# Autodesk Inventor assembly: BowdenDriver
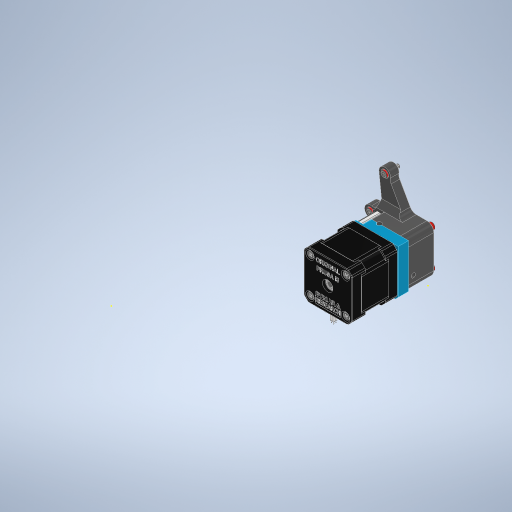
[picture p0: Inventor's stored thumbnail of the model, 512x512]
Saved by Autodesk Inventor 2023 (Build 270158000, 158)
## iProperties
Created: 2023-06-16
Part Number: BowdenDriver
Document SubType Name: Assembly
Designer: Parker
Author: Parker
## Documents named in this file (13)
- D:\000 - PEPCORP CLOUD\00- Legacy\Designs\MK3PRO P1\E2\BowdenDriver.iam
- D:\000 - PEPCORP CLOUD\00- Legacy\Designs\MK3PRO P1\E2\Bowden Back.ipt
- D:\000 - PEPCORP CLOUD\00- Legacy\Designs\MK3PRO P1\E2\E-Motor Mount P1.1.ipt
- D:\000 - PEPCORP CLOUD\00- Legacy\Designs\MK3PRO P1\E2\Extruder Idler V3.ipt
- D:\000 - PEPCORP CLOUD\00- Legacy\Designs\MK3PRO P1\COMPONENTS\NUT_SQUARE_M3.ipt
- D:\000 - PEPCORP CLOUD\00- Legacy\Designs\MK3PRO P1\COMPONENTS\SHCS_M3_40.ipt
- D:\000 - PEPCORP CLOUD\00- Legacy\Designs\MK3PRO P1\COMPONENTS\M3 Washer.ipt
- D:\000 - PEPCORP CLOUD\00- Legacy\Designs\MK3PRO P1\COMPONENTS\Bondtech Idler.ipt
- D:\000 - PEPCORP CLOUD\00- Legacy\Designs\MK3PRO P1\E-Axis\Extruder_stepper_motor V2.iam
- D:\000 - PEPCORP CLOUD\00- Legacy\Designs\MK3PRO P1\COMPONENTS\Bondtech Driver.ipt
- D:\000 - PEPCORP CLOUD\00- Legacy\Designs\MK3PRO P1\COMPONENTS\SHCS_M3_35.ipt
- D:\000 - PEPCORP CLOUD\00- Legacy\Designs\MK3PRO P1\COMPONENTS\SHCS_M3_30.ipt
- D:\000 - PEPCORP CLOUD\00- Legacy\Designs\MK3PRO P1\COMPONENTS\SHCS_M3_8.ipt
## Components (16 placed, 12 different names)
1. Bowden Back:1 — Mate:1, Mate:2, Mate:3, Mate:4, Mate:5, Mate:6, Mate:7, Mate:8, Mate:15, Mate:16, Mate:18, Mate:19, Mate:20, Mate:21, Mate:22, Mate:23, Mate:24, Mate:25, Mate:26, Mate:27, Mate:28, Mate:29
2. E-Motor Mount P1.1:1 — Mate:1, Mate:2, Mate:3, Mate:14
3. Extruder Idler V3:1 — Mate:4, Mate:5, Mate:11, Mate:13, Flush:2
4. NUT_SQUARE_M3:1 — Mate:6, Mate:7, Flush:1
5. SHCS_M3_40:1 — Mate:8, Flush:1, Mate:9, Mate:10, Mate:12
6. M3 Washer:1 — Mate:9, Mate:10
7. M3 Washer:2 — Mate:11, Mate:12
8. Bondtech Idler:1 — Mate:13, Flush:2, Flush:3
9. Extruder_stepper_motor V2:1 [sub-assembly] — Mate:14, Mate:15, Mate:16, Mate:17
10. Bondtech Driver:1 — Mate:17, Flush:3
11. SHCS_M3_35:1 — Mate:20, Mate:22
12. SHCS_M3_35:2 — Mate:19, Mate:21
13. SHCS_M3_35:3 — Mate:18, Mate:23
14. SHCS_M3_30:1 — Mate:24, Mate:25
15. SHCS_M3_8:1 — Mate:26, Mate:29
16. SHCS_M3_8:2 — Mate:27, Mate:28
## Relationships (32: Mate 29, Flush 3)
- Mate:1: Bowden Back:1 ↔ E-Motor Mount P1.1:1
- Mate:2: Bowden Back:1 ↔ E-Motor Mount P1.1:1
- Mate:3: Bowden Back:1 ↔ E-Motor Mount P1.1:1
- Mate:4: Bowden Back:1 ↔ Extruder Idler V3:1
- Mate:5 (0.25 mm): Bowden Back:1 ↔ Extruder Idler V3:1
- Mate:6: Bowden Back:1 ↔ NUT_SQUARE_M3:1
- Mate:7: Bowden Back:1 ↔ NUT_SQUARE_M3:1
- Mate:8: Bowden Back:1 ↔ SHCS_M3_40:1
- Flush:1 (-5 mm): NUT_SQUARE_M3:1 ↔ SHCS_M3_40:1
- Mate:9: SHCS_M3_40:1 ↔ M3 Washer:1
- Mate:10: SHCS_M3_40:1 ↔ M3 Washer:1
- Mate:11: Extruder Idler V3:1 ↔ M3 Washer:2
- Mate:12: SHCS_M3_40:1 ↔ M3 Washer:2
- Mate:13: Extruder Idler V3:1 ↔ Bondtech Idler:1
- Flush:2 (1.5 mm): Extruder Idler V3:1 ↔ Bondtech Idler:1
- Mate:14: E-Motor Mount P1.1:1 ↔ Extruder_stepper_motor V2:1
- Mate:15: Bowden Back:1 ↔ Extruder_stepper_motor V2:1
- Mate:16: Bowden Back:1 ↔ Extruder_stepper_motor V2:1
- Mate:17: Extruder_stepper_motor V2:1 ↔ Bondtech Driver:1
- Flush:3: Bondtech Idler:1 ↔ Bondtech Driver:1
- Mate:18: Bowden Back:1 ↔ SHCS_M3_35:3
- Mate:19: Bowden Back:1 ↔ SHCS_M3_35:2
- Mate:20: Bowden Back:1 ↔ SHCS_M3_35:1
- Mate:21: Bowden Back:1 ↔ SHCS_M3_35:2
- Mate:22: Bowden Back:1 ↔ SHCS_M3_35:1
- Mate:23: Bowden Back:1 ↔ SHCS_M3_35:3
- Mate:24: Bowden Back:1 ↔ SHCS_M3_30:1
- Mate:25: Bowden Back:1 ↔ SHCS_M3_30:1
- Mate:26: Bowden Back:1 ↔ SHCS_M3_8:1
- Mate:27: Bowden Back:1 ↔ SHCS_M3_8:2
- Mate:28: Bowden Back:1 ↔ SHCS_M3_8:2
- Mate:29: Bowden Back:1 ↔ SHCS_M3_8:1
